# Autodesk Inventor assembly: Solar Assembly
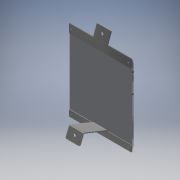
[picture p0: Inventor's stored thumbnail of the model, 180x180]
Saved by Autodesk Inventor 2019 (Build 230136000, 136)
## iProperties
Created: 2020-02-21
Part Number: Solar Assembly
Document SubType Name: Assembly
Designer: gfb14170
Author: gfb14170
## Documents named in this file (4)
- N:\Sandpit\Callum Brooksby\Solar Panel\Solar Assembly.iam
- N:\Sandpit\Callum Brooksby\Solar Panel\Solar Panel.ipt
- N:\Sandpit\Callum Brooksby\Solar Panel\Top Mount.ipt
- N:\Sandpit\Callum Brooksby\Solar Panel\Bottom Mount.ipt
## Components (3 placed, 3 different names)
1. Solar Panel:1 — Flush:1, Mate:2, Insert:1, Flush:2, Mate:4, Insert:2
2. Top Mount:1 — Flush:1, Mate:1, Angle:1, Insert:1
3. Bottom Mount:1 — Flush:2, Mate:3, Angle:2, Insert:2
## Relationships (10: Mate 4, Flush 2, Angle 2, Insert 2)
- Flush:1: Solar Panel:1 ↔ Top Mount:1
- Mate:1: Top Mount:1
- Angle:1 (0 deg): Top Mount:1
- Mate:2: Solar Panel:1
- Insert:1: Solar Panel:1 ↔ Top Mount:1
- Flush:2: Solar Panel:1 ↔ Bottom Mount:1
- Mate:3: Bottom Mount:1
- Angle:2 (0 deg): Bottom Mount:1
- Mate:4: Solar Panel:1
- Insert:2: Solar Panel:1 ↔ Bottom Mount:1
